# Autodesk Inventor assembly: pcb
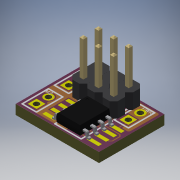
[picture p0: Inventor's stored thumbnail of the model, 180x180]
Saved by Autodesk Inventor 2016 (Build 200138000, 138)
## iProperties
Created: 2015-09-30
Part Number: pcb
Document SubType Name: Assembly
Designer: sawai
Author: sawai
## Documents named in this file (4)
- D:\oneDrive\projects\dualMotorController\cad\pcb.iam
- D:\oneDrive\projects\dualMotorController\cad\assets\pcb.iam
- D:\oneDrive\projects\dualMotorController\cad\soic8.ipt
- D:\oneDrive\projects\dualMotorController\cad\header2x1.ipt
## Components (5 placed, 3 different names)
1. pcb:1 [sub-assembly] — Mate:1, Angle:1, Mate:5
2. soic8:1 — Mate:1, Angle:1
3. header2x1:3 — Mate:3, Flush:2, Flush:3, Flush:4
4. header2x1:4 — Mate:3, Mate:4, Flush:1, Flush:2, Flush:3, Mate:5
5. header2x1:5 — Mate:4, Flush:1, Flush:4
## Relationships (9: Mate 4, Flush 4, Angle 1)
- Mate:1: pcb:1 ↔ soic8:1
- Angle:1 (0 deg): pcb:1 ↔ soic8:1
- Mate:3: header2x1:3 ↔ header2x1:4
- Mate:4: header2x1:4 ↔ header2x1:5
- Flush:1: header2x1:4 ↔ header2x1:5
- Flush:2: header2x1:3 ↔ header2x1:4
- Flush:3: header2x1:3 ↔ header2x1:4
- Flush:4: header2x1:3 ↔ header2x1:5
- Mate:5: pcb:1 ↔ header2x1:4
